# Autodesk Inventor assembly: CDQSB25-40DM(0_1_0)
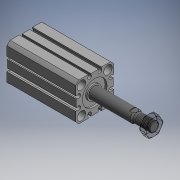
[picture p0: Inventor's stored thumbnail of the model, 180x180]
Saved by Autodesk Inventor 2019.4 (Build 234330000, 330)
## iProperties
Category: PARTsolutions
Company: SMC
Part Number: CDQSB25-40DM(0_1_0)
Catalog Web Link: www.cadenas.de
Description: CQS/CDQS-Compact Cylinder:Standard Type Double Acting,Single Rod
Vendor: SMC
Document SubType Name: Assembly
Designer: partserver
Manufacturer: SMC
Mass: 81.6556 g
Surface Area: 349.207 cm^2
Volume: 81.6556 cm^3
Density: 1 g/cm^3
PSOL_IDENT_0: {$CADENAS_DATA\23d-libs\smc_jp\actuator\compact_cylinder\cqs\cqs_asmtab.prj},301 {VTYP=3D},{STYP=ASS
PSOL_IDENT_1: TAB},{NB=CDQSB25-40DM(0_1_0)},{LINA=CDQSB25-40DM},{NN=CQS/CDQS},{DATE=18.11.2021 10:45:43},{GEOMDATE=
PSOL_IDENT_2: 27.09.2019 04:14:02},{VERSION=},{LINEID=40},{WBVAR=TYPE,MAGNET,AUTOSWITCH,LEAD,NUMBER,STROKE,POS,BOD
PSOL_IDENT_3: Y,STOP,OMSC1,OMSC2,OMSC3,OMSC4,OMSC5,OMSC6,OMSC7,THREAD},{WBNUMERIC=STROKE,POS}  {NB=CDQSB25-40DM(0_
PSOL_IDENT_4: 1_0)},{LINA=CDQSB25-40DM},{KT=DUMMY},{TYPE=},{TYPEX='','(-) None','10-','(10) Relief type','11-','(1
PSOL_IDENT_5: 1) Vacuum type','21-','(21) Copper,fluorine and silicon-free + Low particle generation (Relief type)'
PSOL_IDENT_6: ,'22-', '(22) Copper,fluorine and silicon-free + Low particle generation (Vacuum suction type)'},{BO
PSOL_IDENT_7: RE=25},{MOUNT=(B) Through-hole/Both ends tapped common (Standard)},{MOUNTX=B},{MAGNET=D},{AUTOSWITCH=
PSOL_IDENT_8: },{AUTOSWITCHX='','(-) Without autoswitch','-M9NV','M9NV','-M9PV','M9PV','-M9BV','M9BV','-M9N','M9N'
PSOL_IDENT_9: ,'-M9P','M9P','-M9B','M9B','-M9NWV','M9NWV','-M9PWV','M9PWV','-M9BWV','M9BWV','-M9NW','M9NW','-M9PW'
PSOL_IDENT_10: ,'M9PW','-M9BW','M9BW','-M9NAV','M9NAV','-M9PAV','M9PAV','-M9BAV','M9BAV','-M9NA','M9NA','-M9PA','M9
PSOL_IDENT_11: PA','-M9BA','M9BA','-A96V','A96V','-A93V','A93V','-A90V','A90V','-A96','A96','-A93','A93','-A90','A9
PSOL_IDENT_12: 0','-P3DWA','P3DWA','-P3DWASC','P3DWASC','-P3DWASE','P3DWASE'},{LEAD=},{LEADX='','N/A'},{NUMBER=},{N
PSOL_IDENT_13: UMBERX='','N/A'},{STROKE=40},{STROKEX=[5:300/1]},{SMIN=5},{SMINX=5},{SMAX=300},{POS=0},{ACTION=(D) D
PSOL_IDENT_14: ouble acting},{BODY=M},{BODYX='','(-) Standard (Rod end female thread)','C','(C) With rubber bumper'
PSOL_IDENT_15: ,'M','(M) Rod end male thread','F','(F) Boss on head side','CM','(CM) With rubber bumper & Rod end m
PSOL_IDENT_16: ale thread','FC','(FC) Boss on head side & With rubber bumper','FM','(FM) Boss on head side & Rod en
PSOL_IDENT_17: d male thread','FCM','(FCM) Boss on head side & With rubber bumper & Rod end male thread'},{STOP=1},
PSOL_IDENT_18: {COM=Please confirm the conditions of use with SMC},{STOPX='0','Standard stroke', '1','Manufacturabl
PSOL_IDENT_19: e stroke','2','(-XB10) Intermediate stroke(Exclusive body)'},{OMSC1=},{OMSC1X= '','N/A' },{OMSC2=},{
PSOL_IDENT_20: OMSC2X='','(-) Without order','-XB9','(-XB9) Low speed cylinder (10 to 50 mm/s)','-XB13','(-XB13) Lo
PSOL_IDENT_21: w speed cylinder (5 to 50 mm/s)'},{OMSC3=},{OMSC3X='','(-) Without order','-XC6','(-XC6) Piston rod,
PSOL_IDENT_22: retaining ring, rod end nut made of stainless steel','-X271','(-X271) Fluororubber seals'},{OMSC4=}
PSOL_IDENT_23: ,{OMSC4X='','(-) Without order','-XC36','(-XC36) With boss in rod side'},{OMSC5=},{OMSC5X='','(-) Wi
PSOL_IDENT_24: thout order','-XC85','(-XC85) Grease for food processing equipment'},{OMSC6=},{OMSC6X='','(-) Withou
PSOL_IDENT_25: t order','-X1876','(-X1876) With concave shape end boss on the cylinder tube head side'},{OMSC7=},{O
PSOL_IDENT_26: MSC7X='','N/A'},{THREAD=0},{ORDER=CDQSB25-40DM},{A=37.5},{AA1=27.5},{AA2=37.5},{AA3=59.0},{B=32.5},{
PSOL_IDENT_27: BB1=22.5},{BB2=32.5},{BB3=44.0},{F=5.5},{FF1=5.5},{FF2=5.5},{FF3=11.0},{L=5.0},{LL1=5.0},{LL2=15.0},
PSOL_IDENT_28: {C=12},{D=12},{E=40},{H=M6x1.0},{I=52},{K=10},{M=28.0},{N=5.4},{OA=M6x1.0},{OB=9.0},{Q=11.0},{RA=10}
PSOL_IDENT_29: ,{RB=7},{T=1.0},{B1=17},{C1=15},{H1=6},{L1=22.5},{L11=22.5},{L12=32.5},{MM=M10x1.25},{X=17.5},{LD=0.
PSOL_IDENT_30: 0},{LG=0.0},{LH=0},{LT=0.0},{LX=0.000},{LY=0.0},{LZ=0},{XX=0.0},{Y=0.0},{FD=0.0},{FT=0.0},{FV=0},{FX=
PSOL_IDENT_31: 0},{FZ=0},{CB=0},{CD=0},{CT=0},{CU=0},{CW=0},{CX=0.0},{CZ=0},{RR=0},{OMSCX=},{PPATH=cqs/assembly/cqs
PSOL_IDENT_32: _asmsbl.prj}
NB: CDQSB25-40DM(0_1_0)
NN: CQS/CDQS
NT: Compact Cylinder:Standard Type Double Acting,Single Rod
NBSYN: $ORDER.($POS._$STOP._$THREAD.)
LINA: CDQSB25-40DM
CATALOG: SMC (JP
BORE: 25
MOUNT: (B) Through-hole/Both ends tapped common (Standard)
MAGNET: (D) With magnet
AUTOSWITCH: (-) Without autoswitch
LEAD: N/A
NUMBER: N/A
STROKE: 40
POS: 0
ACTION: (D) Double acting
BODY: (M) Rod end male thread
STOP: Manufacturable stroke
COM: Please confirm the conditions of use with SMC
OMSC1: N/A
OMSC2: (-) Without order
OMSC3: (-) Without order
OMSC4: (-) Without order
OMSC5: (-) Without order
OMSC6: (-) Without order
OMSC7: N/A
THREAD: on
SUPPLIER: SMC
ARTICLENO: CDQSB25-40DM(0_1_0)
BOMINFO: CDQSB25-40DM
CREATOR: CADENAS GmbH
Title: CDQSB25-40DM
Author: Cadenas PARTsolutions
Comments: Compact Cylinder:Standard Type Double Acting,Single Rod
## Documents named in this file (4)
- C:\Users\堀川皓史\Desktop\ロボ研\NHKフォルダ\2022NHKロボコン\R2_version1\AIS2017\CDQSB25-40DM(0_1_0).iam
- C:\Users\堀川皓史\Desktop\ロボ研\NHKフォルダ\2022NHKロボコン\R2_version1\AIS2017\CDQSB25-40DM(1_0)_BODY.ipt
- C:\Users\堀川皓史\Desktop\ロボ研\NHKフォルダ\2022NHKロボコン\R2_version1\AIS2017\CDQSB25-40DM(1_0)_ROD.ipt
- C:\Users\堀川皓史\Desktop\ロボ研\NHKフォルダ\2022NHKロボコン\R2_version1\AIS2017\NT-03_CQS.ipt
## Components (3 placed, 3 different names)
1. CDQSB25-40DM(1_0)_BODY:1 — BODY_ROD_Z@1 <-> ROD_BODY_Z@2, BODY_ROD_YZ@1 <-> ROD_BODY_YZ@2, 円柱状:1
2. CDQSB25-40DM(1_0)_ROD:1 — BODY_ROD_Z@1 <-> ROD_BODY_Z@2, BODY_ROD_YZ@1 <-> ROD_BODY_YZ@2, ROD_NUT_XY@2 <-> NUT_ROD_XY@3, ROD_NUT_Z@2 <-> NUT_ROD_Z@3, ROD_NUT_YZ@2 <-> NUT_ROD_YZ@3, 円柱状:1
3. NT-03_CQS:1 — ROD_NUT_XY@2 <-> NUT_ROD_XY@3, ROD_NUT_Z@2 <-> NUT_ROD_Z@3, ROD_NUT_YZ@2 <-> NUT_ROD_YZ@3
## Relationships (6: Mate 3, Angle 2, CylindricalJoint 1)
- BODY_ROD_Z@1 <-> ROD_BODY_Z@2 [Mate]: CDQSB25-40DM(1_0)_BODY:1 ↔ CDQSB25-40DM(1_0)_ROD:1
- BODY_ROD_YZ@1 <-> ROD_BODY_YZ@2 [Angle] (0 deg): CDQSB25-40DM(1_0)_BODY:1 ↔ CDQSB25-40DM(1_0)_ROD:1
- ROD_NUT_XY@2 <-> NUT_ROD_XY@3 [Mate] (-3 mm): CDQSB25-40DM(1_0)_ROD:1 ↔ NT-03_CQS:1
- ROD_NUT_Z@2 <-> NUT_ROD_Z@3 [Mate]: CDQSB25-40DM(1_0)_ROD:1 ↔ NT-03_CQS:1
- ROD_NUT_YZ@2 <-> NUT_ROD_YZ@3 [Angle] (0 deg): CDQSB25-40DM(1_0)_ROD:1 ↔ NT-03_CQS:1
- 円柱状:1 [CylindricalJoint]: CDQSB25-40DM(1_0)_BODY:1 ↔ CDQSB25-40DM(1_0)_ROD:1
